# Autodesk Inventor assembly: Mount
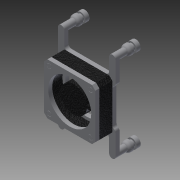
[picture p0: Inventor's stored thumbnail of the model, 180x180]
Saved by Autodesk Inventor 2013 (Build 170138000, 138)
## iProperties
Created: 2014-11-16
Part Number: Mount
Document SubType Name: Assembly
Designer: Kyle
Author: Kyle
## Documents named in this file (5)
- C:\Users\Kyle\Documents\Autodesk\Output\Inventor 2013\Motor Driver Fan Mount\Mount.iam
- C:\Users\Kyle\Documents\Autodesk\Output\Inventor 2013\Motor Driver Fan Mount\Base.ipt
- C:\Users\Kyle\Documents\Autodesk\Output\Inventor 2013\Motor Driver Fan Mount\Fan.ipt
- C:\Users\Kyle\Documents\Autodesk\Output\Inventor 2013\Motor Driver Fan Mount\Cover Plate.ipt
- C:\Users\Kyle\Documents\Autodesk\Output\Inventor 2013\Motor Driver Fan Mount\Mount Pin.ipt
## Components (7 placed, 4 different names)
1. Base:1 — Mate:1, Mate:2, Mate:3, Mate:4, Mate:5, Mate:7, Flush:1, Mate:8, Mate:9, Mate:10, Flush:2, Flush:3, Flush:4
2. Fan:1 — Mate:1, Mate:2, Mate:3, Mate:6
3. Cover Plate:1 — Mate:4, Mate:5, Mate:6
4. Mount Pin:1 — Mate:7, Flush:1
5. Mount Pin:2 — Mate:8, Flush:4
6. Mount Pin:3 — Mate:9, Flush:3
7. Mount Pin:4 — Mate:10, Flush:2
## Relationships (14: Mate 10, Flush 4)
- Mate:1: Base:1 ↔ Fan:1
- Mate:2: Base:1 ↔ Fan:1
- Mate:3: Base:1 ↔ Fan:1
- Mate:4: Base:1 ↔ Cover Plate:1
- Mate:5: Base:1 ↔ Cover Plate:1
- Mate:6: Fan:1 ↔ Cover Plate:1
- Mate:7: Base:1 ↔ Mount Pin:1
- Flush:1: Base:1 ↔ Mount Pin:1
- Mate:8: Base:1 ↔ Mount Pin:2
- Mate:9: Base:1 ↔ Mount Pin:3
- Mate:10: Base:1 ↔ Mount Pin:4
- Flush:2: Base:1 ↔ Mount Pin:4
- Flush:3: Base:1 ↔ Mount Pin:3
- Flush:4: Base:1 ↔ Mount Pin:2
